# Autodesk Inventor assembly: VoltageMonitor
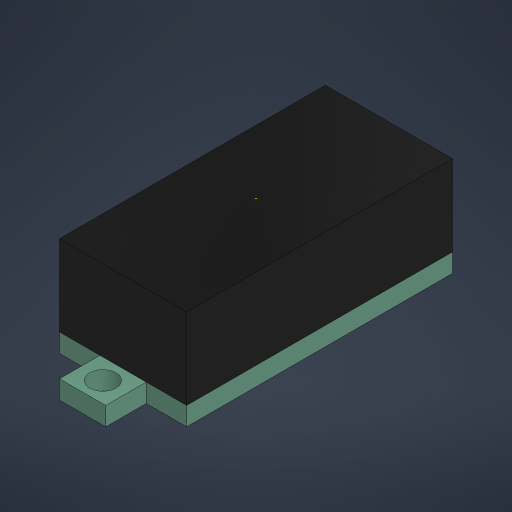
[picture p0: Inventor's stored thumbnail of the model, 512x512]
Saved by Autodesk Inventor 2024.2 (Build 282272000, 272)
## iProperties
Created: 2024-01-12
Part Number: VoltageMonitor
Document SubType Name: Assembly
Designer: Hanaoka
Author: Hanaoka
## Documents named in this file (3)
- G:\共有ドライブ\reRo\05_個人\hanaoka\inventor\PCBs\VoltageMonitor.iam
- G:\共有ドライブ\reRo\05_個人\hanaoka\inventor\PCBs\Sengment.ipt
- G:\共有ドライブ\reRo\05_個人\hanaoka\inventor\PCBs\Segment_PCB.ipt
## Components (2 placed, 2 different names)
1. Sengment:1 — フラッシュ:1, フラッシュ:2
2. Segment_PCB:1 — フラッシュ:1, フラッシュ:2
## Relationships (2: Flush 2)
- フラッシュ:1 [Flush]: Sengment:1 ↔ Segment_PCB:1
- フラッシュ:2 [Flush]: Sengment:1 ↔ Segment_PCB:1
